# Autodesk Inventor assembly: ShootingMechanism
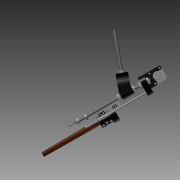
[picture p0: Inventor's stored thumbnail of the model, 180x180]
Saved by Autodesk Inventor 2015 (Build 190159000, 159)
## iProperties
Created: 2017-01-04
Part Number: ShootingMechanism
Document SubType Name: Assembly
Designer: Ernest
Mass: 501.827 g
Surface Area: 1553.31 cm^2
Volume: 501.827 cm^3
Density: 1 g/cm^3
Author: Ernest
## Documents named in this file (21)
- C:\Users\1esh9\Documents\Capstone-Project\doc\CAD\ShootingMechanism\ShootingMechanism.iam
- C:\Users\1esh9\Documents\Capstone-Project\doc\CAD\ShootingMechanism\CueStickTip.ipt
- C:\Users\1esh9\Documents\Capstone-Project\doc\CAD\ShootingMechanism\ThreadedBar.ipt
- C:\Users\1esh9\Documents\Capstone-Project\doc\CAD\ShootingMechanism\SmoothBar.ipt
- C:\Users\1esh9\Documents\Capstone-Project\doc\CAD\ShootingMechanism\ThreadBarNut.ipt
- C:\Users\1esh9\Documents\Capstone-Project\doc\CAD\ShootingMechanism\LinearBearing.ipt
- C:\Users\1esh9\Documents\Capstone-Project\doc\CAD\ShootingMechanism\FrontStopper.ipt
- C:\Users\1esh9\Documents\Capstone-Project\doc\CAD\ShootingMechanism\PulleyScrew.ipt
- C:\Users\1esh9\Documents\Capstone-Project\doc\CAD\ShootingMechanism\PulleyHolder.ipt
- C:\Users\1esh9\Documents\Capstone-Project\doc\CAD\ShootingMechanism\PulleyNut.ipt
- C:\Users\1esh9\Documents\Capstone-Project\doc\CAD\ShootingMechanism\BackStopper.ipt
- C:\Users\1esh9\Documents\Capstone-Project\doc\CAD\ShootingMechanism\Spring.ipt
- C:\Users\1esh9\Documents\Capstone-Project\doc\CAD\ShootingMechanism\MountBar.ipt
- C:\Users\1esh9\Documents\Capstone-Project\doc\CAD\ShootingMechanism\MountB.ipt
- C:\Users\1esh9\Documents\Capstone-Project\doc\CAD\ShootingMechanism\CueHolderTop.ipt
- C:\Users\1esh9\Documents\Capstone-Project\doc\CAD\ShootingMechanism\CueHolderLBBottom.ipt
- C:\Users\1esh9\Documents\Capstone-Project\doc\CAD\ShootingMechanism\CueHolderBottom.ipt
- C:\Users\1esh9\Documents\Capstone-Project\doc\CAD\ShootingMechanism\CueBeltHorder.ipt
- C:\Users\1esh9\Documents\Capstone-Project\doc\CAD\Wheels-Pulleys\Wheel.ipt
- C:\Users\1esh9\Documents\Capstone-Project\doc\CAD\Stepper Motor\NEMA-17\NEMA 17.iam
- C:\Users\1esh9\Documents\Capstone-Project\doc\CAD\Wheels-Pulleys\Pulley5.ipt
## Components (63 placed, 20 different names)
1. CueStickTip:1 — Mate:20, Flush:2
2. ThreadedBar:1 — Mate:6, Mate:7, Mate:10, Mate:11, Flush:6, Flush:7, Mate:77, Mate:78, Mate:149, Mate:150, Mate:152
3. ThreadedBar:2 — Mate:4, Mate:5, Mate:8, Mate:9, Flush:6, Mate:75, Mate:76, Mate:147, Mate:148, Mate:151
4. SmoothBar:1 — Flush:3, Mate:21, Mate:40, Mate:42, Mate:95, Mate:153
5. SmoothBar:2 — Flush:3, Mate:41, Mate:96, Mate:154
6. ThreadBarNut:1 — Mate:9, Mate:45
7. ThreadBarNut:2 — Mate:4, Mate:22
8. ThreadBarNut:3 — Mate:11, Mate:44
9. ThreadBarNut:4 — Mate:6, Mate:25
10. ThreadBarNut:5 — Mate:10, Mate:43
11. ThreadBarNut:6 — Mate:7, Mate:23
12. ThreadBarNut:7 — Mate:8, Mate:46
13. ThreadBarNut:8 — Mate:5, Mate:24
14. LinearBearing:1 — Flush:1, Mate:96, Mate:97, Mate:101
15. LinearBearing:2 — Flush:1, Flush:2, Mate:95, Mate:98, Flush:39
16. FrontStopper:1 — Mate:20, Mate:21, Mate:22, Mate:23, Mate:24, Mate:25, Mate:36, Mate:38, Mate:39, Mate:145, Mate:148, Mate:150
17. PulleyScrew:1 — Mate:27, Mate:28, Mate:29, Mate:138
18. PulleyHolder:1 — Mate:28, Mate:29, Mate:30, Mate:31, Mate:36, Mate:139, Mate:144
19. PulleyNut:1 — Mate:27, Mate:30
20. PulleyScrew:2 — Mate:31, Mate:34, Flush:4, Mate:144, Mate:145
21. PulleyNut:2 — Mate:34, Flush:4
22. BackStopper:1 — Mate:42, Mate:43, Mate:44, Mate:45, Mate:46, Flush:7, Mate:49, Mate:50, Mate:51, Mate:52, Mate:142, Mate:147, Mate:149, Mate:153, Mate:154
23. Spring:1 — Mate:39, Mate:40
24. Spring:2 — Mate:38, Mate:41
25. PulleyScrew:3 — Mate:49, Flush:10, Mate:140
26. PulleyScrew:4 — Mate:51, Flush:9
27. PulleyScrew:5 — Mate:50, Flush:9, Flush:10, Mate:52, Mate:141
28. MountB:1 — Mate:86, Mate:87, Mate:151, Mate:152, Mate:155
29. ThreadBarNut:15 — Mate:76, Flush:15
30. ThreadBarNut:16 — Mate:75, Flush:16
31. ThreadBarNut:17 — Mate:77, Flush:15
32. ThreadBarNut:18 — Mate:78, Flush:16
33. MountBar:2 — Mate:84, Mate:85, Flush:14, Mate:155
34. ThreadBarNut:19 — Mate:84, Mate:87
35. ThreadBarNut:20 — Mate:85, Flush:14, Mate:86
36. CueHolderLBBottom:1 — Mate:97, Flush:19, Flush:41
37. CueHolderLBBottom:2 — Mate:98, Flush:19, Mate:102, Mate:134, Flush:40
38. CueHolderBottom:1 — Mate:103, Mate:104, Mate:105, Mate:135
39. CueHolderTop:1 — Mate:101, Mate:102, Mate:103, Mate:104, Mate:105, Mate:108, Mate:109, Mate:110, Mate:111, Mate:112, Mate:113, Mate:114, Mate:115, Mate:116, Mate:117, Mate:118, Mate:119, Mate:120, Mate:122, Mate:125, Mate:136, Mate:137, Flush:39, Flush:40, Flush:41
40. CueBeltHorder:1 — Mate:108, Mate:109, Mate:110
41. PulleyScrew:6 — Mate:113, Mate:126, Flush:38
42. PulleyScrew:7 — Mate:116, Flush:22, Mate:131
43. PulleyScrew:8 — Mate:112, Flush:28, Mate:122, Mate:124
44. PulleyScrew:9 — Mate:117, Flush:21, Flush:22, Flush:25, Mate:132
45. PulleyScrew:10 — Mate:115, Flush:21, Mate:130
46. PulleyScrew:11 — Mate:118, Flush:23, Mate:128
47. PulleyScrew:12 — Mate:120, Flush:23, Flush:24, Flush:25, Mate:129, Mate:136
48. PulleyScrew:13 — Mate:119, Flush:24, Mate:127
49. PulleyScrew:14 — Mate:114, Mate:133, Flush:38, Mate:137
50. PulleyScrew:15 — Mate:111, Flush:28, Mate:123
51. PulleyNut:3 — Mate:123, Flush:29, Mate:125
52. PulleyNut:4 — Mate:124, Flush:29
53. PulleyNut:5 — Flush:31, Flush:32, Mate:126, Mate:134
54. PulleyNut:6 — Flush:31, Mate:127
55. PulleyNut:7 — Mate:128, Flush:37
56. PulleyNut:8 — Flush:33, Mate:131
57. PulleyNut:9 — Flush:36, Mate:129, Flush:37, Mate:135
58. PulleyNut:10 — Flush:35, Mate:132
59. PulleyNut:11 — Flush:35, Flush:36, Mate:130
60. PulleyNut:12 — Flush:32, Flush:33, Mate:133
61. Wheel:1 — Mate:138, Mate:139
62. NEMA 17:1 [sub-assembly] — Mate:140, Mate:141, Mate:142, Mate:143, Flush:42
63. Pulley5:1 — Mate:143, Flush:42
## Relationships (127: Mate 97, Flush 30)
- Mate:4: ThreadedBar:2 ↔ ThreadBarNut:2
- Mate:5: ThreadedBar:2 ↔ ThreadBarNut:8
- Mate:6: ThreadedBar:1 ↔ ThreadBarNut:4
- Mate:7: ThreadedBar:1 ↔ ThreadBarNut:6
- Mate:8: ThreadedBar:2 ↔ ThreadBarNut:7
- Mate:9: ThreadedBar:2 ↔ ThreadBarNut:1
- Mate:10: ThreadedBar:1 ↔ ThreadBarNut:5
- Mate:11: ThreadedBar:1 ↔ ThreadBarNut:3
- Mate:20: CueStickTip:1 ↔ FrontStopper:1
- Flush:1: LinearBearing:1 ↔ LinearBearing:2
- Flush:2: CueStickTip:1 ↔ LinearBearing:2
- Flush:3: SmoothBar:1 ↔ SmoothBar:2
- Mate:21: SmoothBar:1 ↔ FrontStopper:1
- Mate:22: ThreadBarNut:2 ↔ FrontStopper:1
- Mate:23: ThreadBarNut:6 ↔ FrontStopper:1
- Mate:24: ThreadBarNut:8 ↔ FrontStopper:1
- Mate:25: ThreadBarNut:4 ↔ FrontStopper:1
- Mate:27: PulleyScrew:1 ↔ PulleyNut:1
- Mate:28: PulleyScrew:1 ↔ PulleyHolder:1
- Mate:29: PulleyScrew:1 ↔ PulleyHolder:1
- Mate:30: PulleyHolder:1 ↔ PulleyNut:1
- Mate:31: PulleyHolder:1 ↔ PulleyScrew:2
- Mate:34: PulleyScrew:2 ↔ PulleyNut:2
- Mate:36: FrontStopper:1 ↔ PulleyHolder:1
- Flush:4 (-6.332 mm): PulleyScrew:2 ↔ PulleyNut:2
- Mate:38: FrontStopper:1 ↔ Spring:2
- Mate:39: FrontStopper:1 ↔ Spring:1
- Mate:40: SmoothBar:1 ↔ Spring:1
- Mate:41: SmoothBar:2 ↔ Spring:2
- Mate:42: SmoothBar:1 ↔ BackStopper:1
- Flush:6: ThreadedBar:1 ↔ ThreadedBar:2
- Mate:43: ThreadBarNut:5 ↔ BackStopper:1
- Mate:44: ThreadBarNut:3 ↔ BackStopper:1
- Mate:45: ThreadBarNut:1 ↔ BackStopper:1
- Mate:46: ThreadBarNut:7 ↔ BackStopper:1
- Flush:7 (-10 mm): ThreadedBar:1 ↔ BackStopper:1
- Mate:49: BackStopper:1 ↔ PulleyScrew:3
- Mate:50: BackStopper:1 ↔ PulleyScrew:5
- Mate:51: BackStopper:1 ↔ PulleyScrew:4
- Flush:9: PulleyScrew:4 ↔ PulleyScrew:5
- Flush:10: PulleyScrew:3 ↔ PulleyScrew:5
- Mate:52: BackStopper:1 ↔ PulleyScrew:5
- Mate:75: ThreadedBar:2 ↔ ThreadBarNut:16
- Mate:76: ThreadedBar:2 ↔ ThreadBarNut:15
- Mate:77: ThreadedBar:1 ↔ ThreadBarNut:17
- Mate:78: ThreadedBar:1 ↔ ThreadBarNut:18
- Mate:84: MountBar:2 ↔ ThreadBarNut:19
- Mate:85: MountBar:2 ↔ ThreadBarNut:20
- Flush:14 (0.2 mm): MountBar:2 ↔ ThreadBarNut:20
- Mate:86: MountB:1 ↔ ThreadBarNut:20
- Mate:87: MountB:1 ↔ ThreadBarNut:19
- Flush:15: ThreadBarNut:15 ↔ ThreadBarNut:17
- Flush:16: ThreadBarNut:16 ↔ ThreadBarNut:18
- Mate:95: SmoothBar:1 ↔ LinearBearing:2
- Mate:96: SmoothBar:2 ↔ LinearBearing:1
- Mate:97: LinearBearing:1 ↔ CueHolderLBBottom:1
- Mate:98: LinearBearing:2 ↔ CueHolderLBBottom:2
- Flush:19: CueHolderLBBottom:1 ↔ CueHolderLBBottom:2
- Mate:101: LinearBearing:1 ↔ CueHolderTop:1
- Mate:102: CueHolderLBBottom:2 ↔ CueHolderTop:1
- Mate:103: CueHolderBottom:1 ↔ CueHolderTop:1
- Mate:104: CueHolderBottom:1 ↔ CueHolderTop:1
- Mate:105: CueHolderBottom:1 ↔ CueHolderTop:1
- Mate:108: CueHolderTop:1 ↔ CueBeltHorder:1
- Mate:109: CueHolderTop:1 ↔ CueBeltHorder:1
- Mate:110: CueHolderTop:1 ↔ CueBeltHorder:1
- Mate:111: CueHolderTop:1 ↔ PulleyScrew:15
- Mate:112: CueHolderTop:1 ↔ PulleyScrew:8
- Mate:113: CueHolderTop:1 ↔ PulleyScrew:6
- Mate:114: CueHolderTop:1 ↔ PulleyScrew:14
- Mate:115: CueHolderTop:1 ↔ PulleyScrew:10
- Mate:116: CueHolderTop:1 ↔ PulleyScrew:7
- Mate:117: CueHolderTop:1 ↔ PulleyScrew:9
- Mate:118: CueHolderTop:1 ↔ PulleyScrew:11
- Mate:119: CueHolderTop:1 ↔ PulleyScrew:13
- Mate:120: CueHolderTop:1 ↔ PulleyScrew:12
- Flush:21: PulleyScrew:9 ↔ PulleyScrew:10
- Flush:22: PulleyScrew:7 ↔ PulleyScrew:9
- Flush:23: PulleyScrew:11 ↔ PulleyScrew:12
- Flush:24: PulleyScrew:12 ↔ PulleyScrew:13
- Flush:25: PulleyScrew:9 ↔ PulleyScrew:12
- Flush:28: PulleyScrew:8 ↔ PulleyScrew:15
- Mate:122: CueHolderTop:1 ↔ PulleyScrew:8
- Mate:123: PulleyScrew:15 ↔ PulleyNut:3
- Mate:124: PulleyScrew:8 ↔ PulleyNut:4
- Flush:29: PulleyNut:3 ↔ PulleyNut:4
- Mate:125: CueHolderTop:1 ↔ PulleyNut:3
- Flush:31: PulleyNut:5 ↔ PulleyNut:6
- Flush:32: PulleyNut:5 ↔ PulleyNut:12
- Flush:33: PulleyNut:8 ↔ PulleyNut:12
- Flush:35: PulleyNut:10 ↔ PulleyNut:11
- Flush:36: PulleyNut:9 ↔ PulleyNut:11
- Mate:126: PulleyScrew:6 ↔ PulleyNut:5
- Mate:127: PulleyScrew:13 ↔ PulleyNut:6
- Mate:128: PulleyScrew:11 ↔ PulleyNut:7
- Mate:129: PulleyScrew:12 ↔ PulleyNut:9
- Mate:130: PulleyScrew:10 ↔ PulleyNut:11
- Mate:131: PulleyScrew:7 ↔ PulleyNut:8
- Mate:132: PulleyScrew:9 ↔ PulleyNut:10
- Mate:133: PulleyScrew:14 ↔ PulleyNut:12
- Flush:37: PulleyNut:7 ↔ PulleyNut:9
- Mate:134: CueHolderLBBottom:2 ↔ PulleyNut:5
- Mate:135: CueHolderBottom:1 ↔ PulleyNut:9
- Mate:136: CueHolderTop:1 ↔ PulleyScrew:12
- Flush:38: PulleyScrew:6 ↔ PulleyScrew:14
- Mate:137: CueHolderTop:1 ↔ PulleyScrew:14
- Flush:39: LinearBearing:2 ↔ CueHolderTop:1
- Flush:40: CueHolderLBBottom:2 ↔ CueHolderTop:1
- Flush:41: CueHolderLBBottom:1 ↔ CueHolderTop:1
- Mate:138: PulleyScrew:1 ↔ Wheel:1
- Mate:139 (1.7 mm): PulleyHolder:1 ↔ Wheel:1
- Mate:140: PulleyScrew:3 ↔ NEMA 17:1
- Mate:141: PulleyScrew:5 ↔ NEMA 17:1
- Mate:142: BackStopper:1 ↔ NEMA 17:1
- Mate:143: NEMA 17:1 ↔ Pulley5:1
- Flush:42: NEMA 17:1 ↔ Pulley5:1
- Mate:144: PulleyHolder:1 ↔ PulleyScrew:2
- Mate:145: FrontStopper:1 ↔ PulleyScrew:2
- Mate:147: ThreadedBar:2 ↔ BackStopper:1
- Mate:148: ThreadedBar:2 ↔ FrontStopper:1
- Mate:149: ThreadedBar:1 ↔ BackStopper:1
- Mate:150: ThreadedBar:1 ↔ FrontStopper:1
- Mate:151: ThreadedBar:2 ↔ MountB:1
- Mate:152: ThreadedBar:1 ↔ MountB:1
- Mate:153: SmoothBar:1 ↔ BackStopper:1
- Mate:154: SmoothBar:2 ↔ BackStopper:1
- Mate:155: MountB:1 ↔ MountBar:2
